# Autodesk Inventor assembly: verticalStop
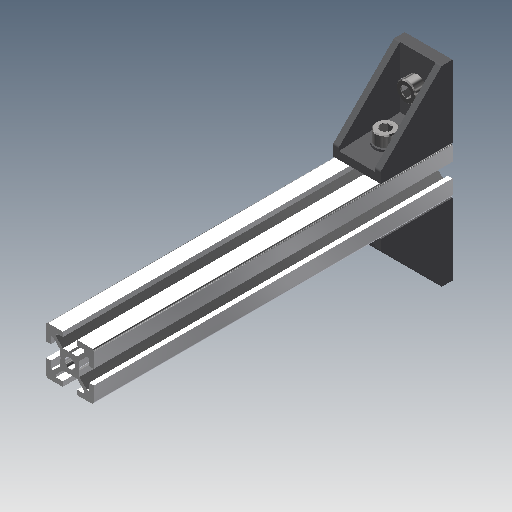
[picture p0: Inventor's stored thumbnail of the model, 512x512]
Saved by Autodesk Inventor 2018 (Build 220112000, 112)
## iProperties
Created: 2017-04-19
Part Number: verticalStop
Document SubType Name: Assembly
Designer: sawaiz
Author: sawaiz
## Documents named in this file (3)
- C:\Users\sawaiz\OneDrive\projects\sPhenixTileTestStand\frame\verticalStop.iam
- C:\Users\sawaiz\OneDrive\projects\sPhenixTileTestStand\frame\hfs5-2020Height.ipt
- C:\Users\sawaiz\OneDrive\projects\sPhenixTileTestStand\hardware\angleBracket.iam
## Components (3 placed, 2 different names)
1. hfs5-2020Height:1 — Mate:1, Flush:1, Flush:2, Mate:2, Flush:3
2. angleBracket:1 [sub-assembly] — Flush:2, Mate:2, Flush:4, Symmetry:1, Symmetry:2
3. angleBracket:2 [sub-assembly] — Mate:1, Flush:1, Flush:3, Flush:4, Symmetry:1, Symmetry:2
## Relationships (8: Flush 4, Mate 2, Symmetry 2)
- Mate:1: hfs5-2020Height:1 ↔ angleBracket:2
- Flush:1: hfs5-2020Height:1 ↔ angleBracket:2
- Flush:2: hfs5-2020Height:1 ↔ angleBracket:1
- Mate:2: hfs5-2020Height:1 ↔ angleBracket:1
- Flush:3: hfs5-2020Height:1 ↔ angleBracket:2
- Flush:4: angleBracket:1 ↔ angleBracket:2
- Symmetry:1: angleBracket:1 ↔ angleBracket:2
- Symmetry:2: angleBracket:1 ↔ angleBracket:2
